# Autodesk Inventor assembly: valve_driver
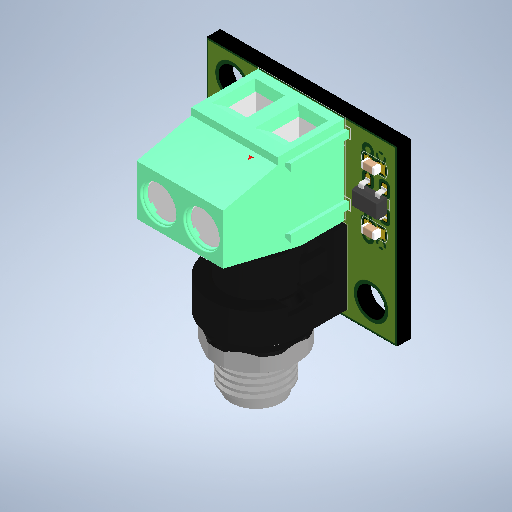
[picture p0: Inventor's stored thumbnail of the model, 512x512]
Saved by Autodesk Inventor 2025.4 (Build 294407000, 407)
## iProperties
Created: 2025-07-29
Part Number: valve_driver
Document SubType Name: Assembly
Designer: Yuhsuan Chen
Author: Yuhsuan Chen
## Documents named in this file (11)
- C:\Users\Yuhsuan Chen\University College London\SWC.Fablab - Documents\swc_fablab_staff\Electronics\Roger\Inventor PRJ New\valve driver\Source\PCBA\valve_driver.iam
- C:\Users\Yuhsuan Chen\University College London\SWC.Fablab - Documents\swc_fablab_staff\Electronics\Roger\Inventor PRJ New\valve driver\Source\PCBA\valve_driver_BOARD.ipt
- C:\Users\Yuhsuan Chen\University College London\SWC.Fablab - Documents\swc_fablab_staff\Electronics\Roger\Inventor PRJ New\valve driver\Source\PCBA\ConvertedComponents\RES_CHIP_0603_CMP-633-0013-26.ipt
- C:\Users\Yuhsuan Chen\University College London\SWC.Fablab - Documents\swc_fablab_staff\Electronics\Roger\Inventor PRJ New\valve driver\Source\PCBA\ConvertedComponents\853-004-213R00Y_CMP-370-0028-8.ipt
- C:\Users\Yuhsuan Chen\University College London\SWC.Fablab - Documents\swc_fablab_staff\Electronics\Roger\Inventor PRJ New\valve driver\Source\PCBA\ConvertedComponents\CAP_CHIP_0805_CMP-611-0000-9.ipt
- C:\Users\Yuhsuan Chen\University College London\SWC.Fablab - Documents\swc_fablab_staff\Electronics\Roger\Inventor PRJ New\valve driver\Source\PCBA\ConvertedComponents\TH-5.00-1X2P_CMP-00028-6.ipt
- C:\Users\Yuhsuan Chen\University College London\SWC.Fablab - Documents\swc_fablab_staff\Electronics\Roger\Inventor PRJ New\valve driver\Source\PCBA\ConvertedComponents\RES_CHIP_0805_CMP-633-0220-1.ipt
- C:\Users\Yuhsuan Chen\University College London\SWC.Fablab - Documents\swc_fablab_staff\Electronics\Roger\Inventor PRJ New\valve driver\Source\PCBA\ConvertedComponents\SOT23-5_CMP-970-0051-1.ipt
- C:\Users\Yuhsuan Chen\University College London\SWC.Fablab - Documents\swc_fablab_staff\Electronics\Roger\Inventor PRJ New\valve driver\Source\PCBA\ConvertedComponents\SOIC8_EP_TI_CMP-970-0052-3.ipt
- C:\Users\Yuhsuan Chen\University College London\SWC.Fablab - Documents\swc_fablab_staff\Electronics\Roger\Inventor PRJ New\valve driver\Source\PCBA\ConvertedComponents\CAP_CHIP_0603_CMP-611-0027-24.ipt
- C:\Users\Yuhsuan Chen\University College London\SWC.Fablab - Documents\swc_fablab_staff\Electronics\Roger\Inventor PRJ New\valve driver\Source\PCBA\ConvertedComponents\pin header\TSW-103-08-L-S-RA.iam
## Components (12 placed, 12 different names)
1. valve_driver_BOARD:1 — Mate:1, Angle:1, Mate:2, Angle:2, Mate:3, Angle:3, Mate:4, Flush:1
2. RES_CHIP_0603_CMP-633-0013-26:1{R1}
3. TH-5.00-1X2P_CMP-00028-6:1{CN3}
4. RES_CHIP_0805_CMP-633-0220-1:1{R2}
5. SOT23-5_CMP-970-0051-1:1{U1}
6. SOIC8_EP_TI_CMP-970-0052-3:1{U2}
7. CAP_CHIP_0603_CMP-611-0027-24:1{C3}
8. CAP_CHIP_0603_CMP-611-0027-24:2{C2}
9. CAP_CHIP_0603_CMP-611-0027-24:3{C1}
10. 853-004-213R00Y_CMP-370-0028-8:1{CN2}
11. CAP_CHIP_0805_CMP-611-0000-9:1{C4}
12. TSW-103-08-L-S-RA:1 [sub-assembly] — Mate:4, Flush:1, Mate:5
## Relationships (9: Mate 5, Angle 3, Flush 1)
- Mate:1: valve_driver_BOARD:1
- Angle:1 (0 deg): valve_driver_BOARD:1
- Mate:2: valve_driver_BOARD:1
- Angle:2 (0 deg): valve_driver_BOARD:1
- Mate:3: valve_driver_BOARD:1
- Angle:3 (0 deg): valve_driver_BOARD:1
- Mate:4: valve_driver_BOARD:1 ↔ TSW-103-08-L-S-RA:1
- Flush:1: valve_driver_BOARD:1 ↔ TSW-103-08-L-S-RA:1
- Mate:5: TSW-103-08-L-S-RA:1
